# Autodesk Inventor assembly: MegahashColdStorage
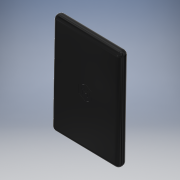
[picture p0: Inventor's stored thumbnail of the model, 180x180]
Saved by Autodesk Inventor 2017 (Build 210142000, 142)
## iProperties
Created: 2018-08-01
Part Number: MegahashColdStorage
Document SubType Name: Assembly
Designer: intelsath
Author: intelsath
## Documents named in this file (20)
- C:\Users\intelsath\Documents\Inventor\Cryptowallet\MegahashColdStorage.iam
- C:\Users\intelsath\Documents\Inventor\Cryptowallet\PCB.ipt
- C:\Users\intelsath\Documents\Inventor\Cryptowallet\micro_usb_connector.iam
- C:\Users\intelsath\Documents\Inventor\Cryptowallet\SiP.ipt
- C:\Users\intelsath\Documents\Inventor\Cryptowallet\0603 LED v7.ipt
- C:\Users\intelsath\Documents\Inventor\Cryptowallet\Battery.ipt
- C:\Users\intelsath\Documents\Inventor\Cryptowallet\Crystal 3225.ipt
- C:\Users\intelsath\Documents\Inventor\Cryptowallet\MicroSD-holder.ipt
- C:\Users\intelsath\Documents\Inventor\Cryptowallet\Pogo-pin.ipt
- C:\Users\intelsath\Documents\Inventor\Cryptowallet\Push-button.ipt
- C:\Users\intelsath\Documents\Inventor\Cryptowallet\QFN-24 3x3 0.4mm.ipt
- C:\Users\intelsath\Documents\Inventor\Cryptowallet\QFN24(4X4).ipt
- C:\Users\intelsath\Documents\Inventor\Cryptowallet\QFN32.ipt
- C:\Users\intelsath\Documents\Inventor\Cryptowallet\SM02B-SRSS-TB.ipt
- C:\Users\intelsath\Documents\Inventor\Cryptowallet\SHR-02V-S-B.ipt
- C:\Users\intelsath\Documents\Inventor\Cryptowallet\LCD-Connector.ipt
- C:\Users\intelsath\Documents\Inventor\Cryptowallet\Casing (Back).ipt
- C:\Users\intelsath\Documents\Inventor\Cryptowallet\LED Pipe.ipt
- C:\Users\intelsath\Documents\Inventor\Cryptowallet\LCD+Cover.ipt
- C:\Users\intelsath\Documents\Inventor\Cryptowallet\Button Cap.ipt
## Components (23 placed, 19 different names)
1. PCB:1 — Flush:1, Mate:1, Mate:2, Flush:2, Flush:3, Tangent:1, Mate:3, Flush:4, Flush:5, Flush:6, Mate:4, Mate:5, Mate:6, Mate:7, Flush:8, Flush:9, Mate:9, Flush:10, Flush:11, Mate:10, Mate:11, Flush:12, Flush:13, Flush:15, Mate:12, Flush:16, Flush:17, Flush:18, Flush:19, Mate:13, Flush:20, Flush:21, Mate:14, Flush:22, Flush:23, Mate:15, Flush:24, Flush:25, Mate:16, Flush:26, Flush:27, Mate:17, Flush:28, Mate:18, Flush:29, Mate:19, Flush:30, Mate:20, Flush:31, Insert:1, Insert:2
2. micro_usb_connector:1 [sub-assembly] — Flush:1, Mate:1, Mate:2
3. SiP:1 — Flush:2, Flush:3, Tangent:1, Mate:8, Flush:7
4. 0603 LED v7:1 — Mate:3, Flush:4, Flush:5
5. Battery:1 — Flush:6, Mate:4, Mate:5
6. Crystal 3225:1 — Mate:6, Flush:8, Flush:9
7. Crystal 3225:2 — Mate:7, Mate:8, Flush:7
8. MicroSD-holder:1 — Mate:9, Flush:10, Flush:11
9. Pogo-pin:1 — Mate:11, Flush:12, Flush:14, Flush:15
10. Pogo-pin:2 — Mate:10, Flush:13, Flush:14
11. Push-button:1 — Mate:12, Flush:16, Flush:17, Mate:23
12. MPU-9250:1 — Flush:18, Flush:19, Mate:13
13. MPU-9250:2 — Flush:22, Flush:23, Mate:15
14. QFN24(4X4):1 — Flush:24, Flush:25, Mate:16
15. QFN32:1 — Flush:20, Flush:21, Mate:14
16. QFN32:2 — Flush:26, Flush:27, Mate:17
17. SM02B-SRSS-TB:1 — Flush:28, Mate:18, Flush:29, Slider:1
18. SHR-02V-S-B:1 — Slider:1
19. LCD-Connector:1 — Mate:19, Flush:30, Mate:20
20. Casing (Back):1 — Flush:31, Insert:1, Insert:2, Rigid:1, Mate:21, Mate:22, Mate:24
21. LED Pipe:1 — Rigid:1
22. LCD+Cover:1 — Mate:21, Mate:22
23. Button Cap:1 — Mate:23, Mate:24
## Relationships (60: Flush 31, Mate 24, Insert 2, Tangent 1, TranslationJoint 1, WeldJoint 1)
- Flush:1 (1.45 mm): PCB:1 ↔ micro_usb_connector:1
- Mate:1: PCB:1 ↔ micro_usb_connector:1
- Mate:2: PCB:1 ↔ micro_usb_connector:1
- Flush:2 (9.6 mm): PCB:1 ↔ SiP:1
- Flush:3: PCB:1 ↔ SiP:1
- Tangent:1: PCB:1 ↔ SiP:1
- Mate:3: PCB:1 ↔ 0603 LED v7:1
- Flush:4 (4 mm): PCB:1 ↔ 0603 LED v7:1
- Flush:5 (38.9 mm): PCB:1 ↔ 0603 LED v7:1
- Flush:6: PCB:1 ↔ Battery:1
- Mate:4: PCB:1 ↔ Battery:1
- Mate:5: PCB:1 ↔ Battery:1
- Mate:6: PCB:1 ↔ Crystal 3225:1
- Mate:7: PCB:1 ↔ Crystal 3225:2
- Mate:8 (0.55 mm): SiP:1 ↔ Crystal 3225:2
- Flush:7 (4.2 mm): SiP:1 ↔ Crystal 3225:2
- Flush:8 (35 mm): PCB:1 ↔ Crystal 3225:1
- Flush:9 (2.1 mm): PCB:1 ↔ Crystal 3225:1
- Mate:9: PCB:1 ↔ MicroSD-holder:1
- Flush:10 (1.3 mm): PCB:1 ↔ MicroSD-holder:1
- Flush:11 (1.05 mm): PCB:1 ↔ MicroSD-holder:1
- Mate:10: PCB:1 ↔ Pogo-pin:2
- Mate:11: PCB:1 ↔ Pogo-pin:1
- Flush:12 (6.4 mm): PCB:1 ↔ Pogo-pin:1
- Flush:13 (9.6 mm): PCB:1 ↔ Pogo-pin:2
- Flush:14: Pogo-pin:1 ↔ Pogo-pin:2
- Flush:15 (24.6 mm): PCB:1 ↔ Pogo-pin:1
- Mate:12: PCB:1 ↔ Push-button:1
- Flush:16 (1.66 mm): PCB:1 ↔ Push-button:1
- Flush:17 (6.2 mm): PCB:1 ↔ Push-button:1
- Flush:18 (5.9 mm): PCB:1 ↔ MPU-9250:1
- Flush:19 (5.7 mm): PCB:1 ↔ MPU-9250:1
- Mate:13: PCB:1 ↔ MPU-9250:1
- Flush:20 (3.85 mm): PCB:1 ↔ QFN32:1
- Flush:21 (10 mm): PCB:1 ↔ QFN32:1
- Mate:14: PCB:1 ↔ QFN32:1
- Flush:22 (27.65 mm): PCB:1 ↔ MPU-9250:2
- Flush:23 (3 mm): PCB:1 ↔ MPU-9250:2
- Mate:15: PCB:1 ↔ MPU-9250:2
- Flush:24 (33.15 mm): PCB:1 ↔ QFN24(4X4):1
- Flush:25 (3 mm): PCB:1 ↔ QFN24(4X4):1
- Mate:16: PCB:1 ↔ QFN24(4X4):1
- Flush:26 (33 mm): PCB:1 ↔ QFN32:2
- Flush:27 (5.35 mm): PCB:1 ↔ QFN32:2
- Mate:17: PCB:1 ↔ QFN32:2
- Flush:28 (47.6 mm): PCB:1 ↔ SM02B-SRSS-TB:1
- Mate:18: PCB:1 ↔ SM02B-SRSS-TB:1
- Flush:29 (17.85 mm): PCB:1 ↔ SM02B-SRSS-TB:1
- Slider:1 [TranslationJoint] (0.03 mm): SM02B-SRSS-TB:1 ↔ SHR-02V-S-B:1
- Mate:19: PCB:1 ↔ LCD-Connector:1
- Flush:30 (2.9 mm): PCB:1 ↔ LCD-Connector:1
- Mate:20: PCB:1 ↔ LCD-Connector:1
- Flush:31: PCB:1 ↔ Casing (Back):1
- Insert:1: PCB:1 ↔ Casing (Back):1
- Insert:2: PCB:1 ↔ Casing (Back):1
- Rigid:1 [WeldJoint] (2 mm): Casing (Back):1 ↔ LED Pipe:1
- Mate:21: Casing (Back):1 ↔ LCD+Cover:1
- Mate:22: Casing (Back):1 ↔ LCD+Cover:1
- Mate:23: Push-button:1 ↔ Button Cap:1
- Mate:24: Casing (Back):1 ↔ Button Cap:1
